# Autodesk Inventor assembly: CarrierOld
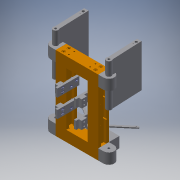
[picture p0: Inventor's stored thumbnail of the model, 180x180]
Saved by Autodesk Inventor 2019 (Build 230136000, 136)
## iProperties
Created: 2019-09-29
Part Number: CarrierOld
Document SubType Name: Assembly
Designer: james
Author: james
## Documents named in this file (10)
- F:\JimsDesign\Jims2020FTC\CarrierOld.iam
- F:\JimsDesign\Jims2020FTC\CarrierBeam.ipt
- F:\JimsDesign\Jims2020FTC\ElvatorEnd.iam
- F:\JimsDesign\Jims2020FTC\SliderRight.iam
- F:\JimsDesign\Jims2020FTC\SliderLeft.iam
- F:\JimsDesign\Jims2020FTC\Hinge.ipt
- F:\JimsDesign\Jims2020FTC\Gripper.ipt
- F:\JimsDesign\Jims2020FTC\ServoBlock.ipt
- F:\JimsDesign\Jims2020FTC\ServoDisk.ipt
- F:\JimsDesign\Jims2020FTC\Arms.ipt
## Components (18 placed, 9 different names)
1. CarrierBeam:1 — Mate:1, Flush:2, Mate:3, Mate:5, Flush:3, Mate:6, Mate:13, Mate:14, Mate:15, Mate:16, Mate:17, Mate:18, Mate:19, Mate:20, Flush:8, Flush:9
2. CarrierBeam:2 — Mate:2, Flush:1, Mate:4, Mate:7, Mate:8, Mate:9, Mate:10, Mate:11, Mate:12, Flush:4, Flush:5, Flush:7, Mate:22, Flush:10, Flush:11, Flush:20
3. ElvatorEnd:1 [sub-assembly] — Mate:1, Mate:2, Flush:1, Flush:2, Mate:3, Mate:4, Flush:14, Flush:15, Mate:23, Flush:19
4. ElvatorEnd:2 [sub-assembly] — Mate:5, Flush:3, Mate:6, Flush:12, Flush:13, Mate:26, Flush:17
5. SliderRight:1 [sub-assembly] — Mate:13, Mate:14, Mate:15
6. SliderRight:2 [sub-assembly] — Mate:16, Mate:17, Mate:18
7. SliderLeft:1 [sub-assembly] — Mate:7, Mate:8, Mate:9
8. SliderLeft:2 [sub-assembly] — Mate:10, Mate:11, Mate:12
9. Hinge:1 — Flush:4, Mate:19, Flush:8, Flush:15
10. Hinge:2 — Flush:5, Mate:20, Flush:9, Flush:12, Mate:25
11. Hinge:3 — Flush:11, Flush:14, Mate:23
12. Hinge:4 — Flush:7, Mate:22, Flush:10, Flush:13, Mate:24
13. Gripper:1 — Mate:24, Flush:16, Mate:34
14. Gripper:2 — Mate:25, Flush:16, Flush:19, Mate:33
15. ServoBlock:1 — Mate:26, Flush:17, Mate:27, Mate:28, Flush:20
16. ServoDisk:1 — Mate:27, Mate:28, Mate:29, Mate:30, Mate:31, Mate:32
17. Arms:1 — Mate:29, Mate:31, Mate:33
18. Arms:2 — Mate:30, Mate:32, Mate:34
## Relationships (51: Mate 33, Flush 18)
- Mate:1: CarrierBeam:1 ↔ ElvatorEnd:1
- Mate:2: CarrierBeam:2 ↔ ElvatorEnd:1
- Flush:1: CarrierBeam:2 ↔ ElvatorEnd:1
- Flush:2: CarrierBeam:1 ↔ ElvatorEnd:1
- Mate:3: CarrierBeam:1 ↔ ElvatorEnd:1
- Mate:4: CarrierBeam:2 ↔ ElvatorEnd:1
- Mate:5: CarrierBeam:1 ↔ ElvatorEnd:2
- Flush:3: CarrierBeam:1 ↔ ElvatorEnd:2
- Mate:6: CarrierBeam:1 ↔ ElvatorEnd:2
- Mate:7: CarrierBeam:2 ↔ SliderLeft:1
- Mate:8: CarrierBeam:2 ↔ SliderLeft:1
- Mate:9: CarrierBeam:2 ↔ SliderLeft:1
- Mate:10: CarrierBeam:2 ↔ SliderLeft:2
- Mate:11: CarrierBeam:2 ↔ SliderLeft:2
- Mate:12: CarrierBeam:2 ↔ SliderLeft:2
- Mate:13: CarrierBeam:1 ↔ SliderRight:1
- Mate:14: CarrierBeam:1 ↔ SliderRight:1
- Mate:15: CarrierBeam:1 ↔ SliderRight:1
- Mate:16: CarrierBeam:1 ↔ SliderRight:2
- Mate:17: CarrierBeam:1 ↔ SliderRight:2
- Mate:18: CarrierBeam:1 ↔ SliderRight:2
- Flush:4: CarrierBeam:2 ↔ Hinge:1
- Flush:5: CarrierBeam:2 ↔ Hinge:2
- Flush:7: CarrierBeam:2 ↔ Hinge:4
- Mate:19: CarrierBeam:1 ↔ Hinge:1
- Mate:20: CarrierBeam:1 ↔ Hinge:2
- Mate:22: CarrierBeam:2 ↔ Hinge:4
- Flush:8: CarrierBeam:1 ↔ Hinge:1
- Flush:9: CarrierBeam:1 ↔ Hinge:2
- Flush:10: CarrierBeam:2 ↔ Hinge:4
- Flush:11: CarrierBeam:2 ↔ Hinge:3
- Flush:12: ElvatorEnd:2 ↔ Hinge:2
- Flush:13: ElvatorEnd:2 ↔ Hinge:4
- Flush:14: ElvatorEnd:1 ↔ Hinge:3
- Flush:15: ElvatorEnd:1 ↔ Hinge:1
- Mate:23: ElvatorEnd:1 ↔ Hinge:3
- Mate:24: Hinge:4 ↔ Gripper:1
- Mate:25: Hinge:2 ↔ Gripper:2
- Flush:16: Gripper:1 ↔ Gripper:2
- Mate:26: ElvatorEnd:2 ↔ ServoBlock:1
- Flush:17: ElvatorEnd:2 ↔ ServoBlock:1
- Flush:19 (-31.75 mm): ElvatorEnd:1 ↔ Gripper:2
- Mate:27: ServoBlock:1 ↔ ServoDisk:1
- Mate:28: ServoBlock:1 ↔ ServoDisk:1
- Flush:20: CarrierBeam:2 ↔ ServoBlock:1
- Mate:29: ServoDisk:1 ↔ Arms:1
- Mate:30: ServoDisk:1 ↔ Arms:2
- Mate:31: ServoDisk:1 ↔ Arms:1
- Mate:32: ServoDisk:1 ↔ Arms:2
- Mate:33: Gripper:2 ↔ Arms:1
- Mate:34: Gripper:1 ↔ Arms:2
